# Autodesk Inventor assembly: xy_assembly
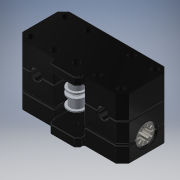
[picture p0: Inventor's stored thumbnail of the model, 180x180]
Saved by Autodesk Inventor 2018 (Build 220112000, 112)
## iProperties
Created: 2018-06-03
Part Number: xy_assembly
Document SubType Name: Assembly
Designer: Z. Deniz
Author: Z. Deniz
## Documents named in this file (6)
- C:\Users\zdeni\Desktop\my3D\3D_Model_v2\montajlar\xy_assembly.iam
- C:\Users\zdeni\Desktop\my3D\3D_Model_v2\parçalar\xy_joint_top.ipt
- C:\Users\zdeni\Desktop\my3D\3D_Model_v2\parçalar\modeller\123RJ4JP_01_08_1.ipt
- C:\Users\zdeni\Desktop\my3D\3D_Model_v2\parçalar\xy_joint_mid.ipt
- C:\Users\zdeni\Desktop\my3D\3D_Model_v2\parçalar\xy_joint_bottom.ipt
- C:\Users\zdeni\Desktop\my3D\3D_Model_v2\parçalar\02131021795.ipt
## Components (8 placed, 5 different names)
1. xy_joint_top:1 — Tangent:1, Mate:1, Mate:2, Tangent:2, Flush:1, Flush:2, Flush:3, Flush:4, Flush:7, Insert:1
2. 123RJ4JP_01_08_1:1 — Mate:2, Tangent:2, Mate:4
3. 123RJ4JP_01_08_1:2 — Tangent:1, Mate:1, Mate:3
4. xy_joint_mid:1 — Flush:1, Mate:3, Flush:2, Mate:5, Flush:7, Mate:6, Flush:9
5. xy_joint_mid:2 — Mate:4, Flush:3, Flush:4, Mate:7
6. xy_joint_bottom:1 — Mate:5, Insert:2, Mate:6, Flush:9, Mate:7
7. 02131021795:1 — Insert:1
8. 02131021795:2 — Insert:2
## Relationships (17: Mate 7, Flush 6, Tangent 2, Insert 2)
- Tangent:1: xy_joint_top:1 ↔ 123RJ4JP_01_08_1:2
- Mate:1: xy_joint_top:1 ↔ 123RJ4JP_01_08_1:2
- Mate:2: xy_joint_top:1 ↔ 123RJ4JP_01_08_1:1
- Tangent:2: xy_joint_top:1 ↔ 123RJ4JP_01_08_1:1
- Flush:1: xy_joint_top:1 ↔ xy_joint_mid:1
- Mate:3: 123RJ4JP_01_08_1:2 ↔ xy_joint_mid:1
- Flush:2: xy_joint_top:1 ↔ xy_joint_mid:1
- Mate:4: 123RJ4JP_01_08_1:1 ↔ xy_joint_mid:2
- Flush:3: xy_joint_top:1 ↔ xy_joint_mid:2
- Flush:4: xy_joint_top:1 ↔ xy_joint_mid:2
- Mate:5: xy_joint_mid:1 ↔ xy_joint_bottom:1
- Flush:7: xy_joint_top:1 ↔ xy_joint_mid:1
- Insert:1 (17.724 mm): xy_joint_top:1 ↔ 02131021795:1
- Insert:2 (-7.405 mm): xy_joint_bottom:1 ↔ 02131021795:2
- Mate:6: xy_joint_mid:1 ↔ xy_joint_bottom:1
- Flush:9: xy_joint_mid:1 ↔ xy_joint_bottom:1
- Mate:7: xy_joint_mid:2 ↔ xy_joint_bottom:1
